# Autodesk Inventor assembly: Assembly2
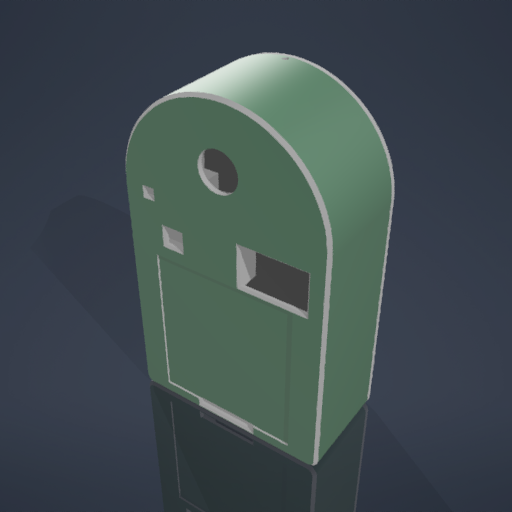
[picture p0: Inventor's stored thumbnail of the model, 512x512]
Saved by Autodesk Inventor 2026.1 (Build 301233020, 233B)
## iProperties
Created: 2025-12-09
Part Number: Assembly2
Document SubType Name: Assembly
Designer: ASUS
Author: ASUS
## Documents named in this file (3)
- C:\Users\ASUS\Documents\Projects\DR DINA DL\Assembly2.iam
- C:\Users\ASUS\Documents\Projects\DR DINA DL\lid.ipt
- C:\Users\ASUS\Documents\Projects\DR DINA DL\enclouser.ipt
## Components (2 placed, 2 different names)
1. lid:1 — Mate:1, Insert:1
2. enclouser:1 — Mate:1, Insert:1
## Relationships (2: Mate 1, Insert 1)
- Mate:1: lid:1 ↔ enclouser:1
- Insert:1: lid:1 ↔ enclouser:1
## Named parameters: Finish1_Area = 458.677, Finish2_Area = 130.596, Finish3_Area = 50.6
note: some values were not read from the file. Shown as the stored number, unit unknown: "Finish1_Area", "Finish2_Area", "Finish3_Area".
